# Autodesk Inventor assembly: TomatoArm1
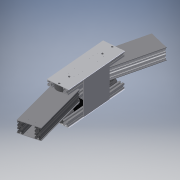
[picture p0: Inventor's stored thumbnail of the model, 180x180]
Saved by Autodesk Inventor 2016 (Build 200138000, 138)
## iProperties
Created: 2016-06-28
Part Number: TomatoArm1
Material: 一般
Document SubType Name: Assembly
Designer: 宏太
Author: 宏太
## Documents named in this file (14)
- C:\Users\宏太\Documents\GitHub\Tomato2016\TomatoArm1.iam
- C:\Users\宏太\Documents\GitHub\Tomato2016\NFS5-2020-260.ipt
- C:\Users\宏太\Documents\GitHub\Tomato2016\bottom_board.ipt
- C:\Users\宏太\Documents\GitHub\Tomato2016\shaft2016.ipt
- C:\Users\宏太\Documents\GitHub\Tomato2016\Servo.iam
- C:\Users\宏太\Documents\GitHub\Tomato2016\BGCSB12\BGCSB12.iam
- C:\Users\宏太\Documents\GitHub\Tomato2016\GEAHBB1.0-40-6-A-10\GEAHBB1_0-40-6-A-10.iam
- C:\Users\宏太\Documents\GitHub\Tomato2016\GEAHBB1.0-40-6-B-10\GEAHBB1_0-40-6-B-10.iam
- C:\Users\宏太\Documents\GitHub\Tomato2016\STHCBT15-MB.iam
- C:\Users\宏太\Documents\GitHub\Tomato2016\Force_Arm_board.ipt
- C:\Users\宏太\Documents\GitHub\Tomato2016\NFS5-2020-230.ipt
- C:\Users\宏太\Documents\GitHub\Tomato2016\sholder_fin.ipt
- C:\Users\宏太\Documents\GitHub\Tomato2016\NFS5-2020-200.ipt
- C:\Users\宏太\Documents\GitHub\Tomato2016\Side_board.ipt
## Components (36 placed, 13 different names)
1. bottom_board:2 — 挿入:1, 挿入:2, 挿入:3, 挿入:4, 挿入:5, 挿入:6, メイト:3, フラッシュ:3, フラッシュ:4, フラッシュ:5, メイト:4, フラッシュ:6, メイト:15, フラッシュ:29, フラッシュ:30, メイト:16, フラッシュ:31, フラッシュ:32
2. Servo:1 [sub-assembly] — 挿入:4, 挿入:9
3. Servo:2 [sub-assembly] — 挿入:3, 挿入:11
4. BGCSB12:1 [sub-assembly] — 挿入:21, 挿入:23, 挿入:24
5. BGCSB12:2 [sub-assembly] — 挿入:22, 挿入:25
6. BGCSB12:3 [sub-assembly] — 挿入:5, 挿入:6, 挿入:7
7. BGCSB12:4 [sub-assembly] — 挿入:1, 挿入:2, 挿入:8
8. GEAHBB1_0-40-6-A-10:1 [sub-assembly] — 挿入:9
9. GEAHBB1_0-40-6-A-10:2 [sub-assembly] — 挿入:11
10. GEAHBB1_0-40-6-B-10:1 [sub-assembly] — 挿入:10
11. GEAHBB1_0-40-6-B-10:2 [sub-assembly] — 挿入:12
12. shaft2016:1 — 挿入:8, 挿入:12, 挿入:13, 挿入:15, 挿入:22
13. shaft2016:2 — 挿入:7, 挿入:10, 挿入:14, 挿入:16, 挿入:21
14. NFS5-2020-260:1 — メイト:3, フラッシュ:3, フラッシュ:4
15. NFS5-2020-260:2 — フラッシュ:5, メイト:4, フラッシュ:6
16. bottom_board:3 — 挿入:23, 挿入:24, 挿入:25, メイト:9, フラッシュ:16, フラッシュ:17, フラッシュ:18, フラッシュ:19, メイト:10
17. STHCBT15-MB:1 [sub-assembly] — 挿入:13, 挿入:17, 挿入:18
18. STHCBT15-MB:2 [sub-assembly] — 挿入:14, 挿入:26, 挿入:27
19. STHCBT15-MB:3 [sub-assembly] — 挿入:16, 挿入:28, 挿入:29
20. STHCBT15-MB:4 [sub-assembly] — 挿入:15, 挿入:19, 挿入:20
21. Force_Arm_board:1 — 挿入:19, 挿入:20, メイト:7, フラッシュ:11, フラッシュ:12, メイト:8, フラッシュ:13, フラッシュ:14
22. Force_Arm_board:2 — 挿入:17, 挿入:18, フラッシュ:7, フラッシュ:8, メイト:5, フラッシュ:9, フラッシュ:10, メイト:6
23. NFS5-2020-230:1 — フラッシュ:9, フラッシュ:10, メイト:6, フラッシュ:15
24. NFS5-2020-230:2 — フラッシュ:7, フラッシュ:8, メイト:5
25. NFS5-2020-230:3 — メイト:7, フラッシュ:11, フラッシュ:12
26. NFS5-2020-230:4 — メイト:8, フラッシュ:13, フラッシュ:14, フラッシュ:15
27. NFS5-2020-260:3 — フラッシュ:18, フラッシュ:19, メイト:10
28. NFS5-2020-260:4 — メイト:9, フラッシュ:16, フラッシュ:17
29. sholder_fin:1 — 挿入:28, 挿入:29, メイト:13, フラッシュ:24, フラッシュ:25, メイト:14, フラッシュ:26, フラッシュ:27
30. sholder_fin:2 — 挿入:26, 挿入:27, メイト:11, フラッシュ:20, フラッシュ:21, フラッシュ:22, メイト:12, フラッシュ:23
31. NFS5-2020-200:1 — メイト:11, フラッシュ:20, フラッシュ:21, フラッシュ:28
32. NFS5-2020-200:2 — メイト:13, フラッシュ:24, フラッシュ:25
33. NFS5-2020-200:3 — メイト:14, フラッシュ:26, フラッシュ:27, フラッシュ:28
34. NFS5-2020-200:4 — フラッシュ:22, メイト:12, フラッシュ:23
35. Side_board:1 — メイト:15, フラッシュ:29, フラッシュ:30
36. Side_board:2 — メイト:16, フラッシュ:31, フラッシュ:32
## Relationships (73: Flush 30, Insert 29, Mate 14)
- 挿入:1 [Insert]: bottom_board:2 ↔ BGCSB12:4
- 挿入:2 [Insert]: bottom_board:2 ↔ BGCSB12:4
- 挿入:3 [Insert]: bottom_board:2 ↔ Servo:2
- 挿入:4 [Insert]: bottom_board:2 ↔ Servo:1
- 挿入:5 [Insert]: bottom_board:2 ↔ BGCSB12:3
- 挿入:6 [Insert]: bottom_board:2 ↔ BGCSB12:3
- 挿入:7 [Insert]: BGCSB12:3 ↔ shaft2016:2
- 挿入:8 [Insert]: BGCSB12:4 ↔ shaft2016:1
- 挿入:9 [Insert]: Servo:1 ↔ GEAHBB1_0-40-6-A-10:1
- 挿入:10 [Insert] (61.5 mm): GEAHBB1_0-40-6-B-10:1 ↔ shaft2016:2
- 挿入:11 [Insert]: Servo:2 ↔ GEAHBB1_0-40-6-A-10:2
- 挿入:12 [Insert] (61.5 mm): GEAHBB1_0-40-6-B-10:2 ↔ shaft2016:1
- メイト:3 [Mate]: bottom_board:2 ↔ NFS5-2020-260:1
- フラッシュ:3 [Flush]: bottom_board:2 ↔ NFS5-2020-260:1
- フラッシュ:4 [Flush] (2 mm): bottom_board:2 ↔ NFS5-2020-260:1
- フラッシュ:5 [Flush]: bottom_board:2 ↔ NFS5-2020-260:2
- メイト:4 [Mate]: bottom_board:2 ↔ NFS5-2020-260:2
- フラッシュ:6 [Flush] (2 mm): bottom_board:2 ↔ NFS5-2020-260:2
- 挿入:13 [Insert] (30 mm): shaft2016:1 ↔ STHCBT15-MB:1
- 挿入:14 [Insert] (30 mm): shaft2016:2 ↔ STHCBT15-MB:2
- 挿入:15 [Insert] (-30 mm): shaft2016:1 ↔ STHCBT15-MB:4
- 挿入:16 [Insert] (-30 mm): shaft2016:2 ↔ STHCBT15-MB:3
- 挿入:17 [Insert]: STHCBT15-MB:1 ↔ Force_Arm_board:2
- 挿入:18 [Insert]: STHCBT15-MB:1 ↔ Force_Arm_board:2
- 挿入:19 [Insert]: STHCBT15-MB:4 ↔ Force_Arm_board:1
- 挿入:20 [Insert]: STHCBT15-MB:4 ↔ Force_Arm_board:1
- フラッシュ:7 [Flush]: Force_Arm_board:2 ↔ NFS5-2020-230:2
- フラッシュ:8 [Flush] (2 mm): Force_Arm_board:2 ↔ NFS5-2020-230:2
- メイト:5 [Mate]: Force_Arm_board:2 ↔ NFS5-2020-230:2
- フラッシュ:9 [Flush] (2 mm): Force_Arm_board:2 ↔ NFS5-2020-230:1
- フラッシュ:10 [Flush]: Force_Arm_board:2 ↔ NFS5-2020-230:1
- メイト:6 [Mate]: Force_Arm_board:2 ↔ NFS5-2020-230:1
- 挿入:21 [Insert]: BGCSB12:1 ↔ shaft2016:2
- 挿入:22 [Insert]: BGCSB12:2 ↔ shaft2016:1
- メイト:7 [Mate]: Force_Arm_board:1 ↔ NFS5-2020-230:3
- フラッシュ:11 [Flush]: Force_Arm_board:1 ↔ NFS5-2020-230:3
- フラッシュ:12 [Flush] (2 mm): Force_Arm_board:1 ↔ NFS5-2020-230:3
- メイト:8 [Mate]: Force_Arm_board:1 ↔ NFS5-2020-230:4
- フラッシュ:13 [Flush]: Force_Arm_board:1 ↔ NFS5-2020-230:4
- フラッシュ:14 [Flush] (2 mm): Force_Arm_board:1 ↔ NFS5-2020-230:4
- フラッシュ:15 [Flush]: NFS5-2020-230:1 ↔ NFS5-2020-230:4
- 挿入:23 [Insert]: BGCSB12:1 ↔ bottom_board:3
- 挿入:24 [Insert]: BGCSB12:1 ↔ bottom_board:3
- 挿入:25 [Insert]: BGCSB12:2 ↔ bottom_board:3
- メイト:9 [Mate]: bottom_board:3 ↔ NFS5-2020-260:4
- フラッシュ:16 [Flush] (2 mm): bottom_board:3 ↔ NFS5-2020-260:4
- フラッシュ:17 [Flush]: bottom_board:3 ↔ NFS5-2020-260:4
- フラッシュ:18 [Flush] (2 mm): bottom_board:3 ↔ NFS5-2020-260:3
- フラッシュ:19 [Flush]: bottom_board:3 ↔ NFS5-2020-260:3
- メイト:10 [Mate]: bottom_board:3 ↔ NFS5-2020-260:3
- 挿入:26 [Insert]: STHCBT15-MB:2 ↔ sholder_fin:2
- 挿入:27 [Insert]: STHCBT15-MB:2 ↔ sholder_fin:2
- 挿入:28 [Insert]: STHCBT15-MB:3 ↔ sholder_fin:1
- 挿入:29 [Insert]: STHCBT15-MB:3 ↔ sholder_fin:1
- メイト:11 [Mate]: sholder_fin:2 ↔ NFS5-2020-200:1
- フラッシュ:20 [Flush]: sholder_fin:2 ↔ NFS5-2020-200:1
- フラッシュ:21 [Flush] (2 mm): sholder_fin:2 ↔ NFS5-2020-200:1
- フラッシュ:22 [Flush]: sholder_fin:2 ↔ NFS5-2020-200:4
- メイト:12 [Mate]: sholder_fin:2 ↔ NFS5-2020-200:4
- フラッシュ:23 [Flush] (2 mm): sholder_fin:2 ↔ NFS5-2020-200:4
- メイト:13 [Mate]: sholder_fin:1 ↔ NFS5-2020-200:2
- フラッシュ:24 [Flush]: sholder_fin:1 ↔ NFS5-2020-200:2
- フラッシュ:25 [Flush] (2 mm): sholder_fin:1 ↔ NFS5-2020-200:2
- メイト:14 [Mate]: sholder_fin:1 ↔ NFS5-2020-200:3
- フラッシュ:26 [Flush]: sholder_fin:1 ↔ NFS5-2020-200:3
- フラッシュ:27 [Flush] (2 mm): sholder_fin:1 ↔ NFS5-2020-200:3
- フラッシュ:28 [Flush]: NFS5-2020-200:1 ↔ NFS5-2020-200:3
- メイト:15 [Mate]: bottom_board:2 ↔ Side_board:1
- フラッシュ:29 [Flush]: bottom_board:2 ↔ Side_board:1
- フラッシュ:30 [Flush] (70 mm): bottom_board:2 ↔ Side_board:1
- メイト:16 [Mate]: bottom_board:2 ↔ Side_board:2
- フラッシュ:31 [Flush]: bottom_board:2 ↔ Side_board:2
- フラッシュ:32 [Flush] (70 mm): bottom_board:2 ↔ Side_board:2
